# Autodesk Inventor assembly: Soporte filamento
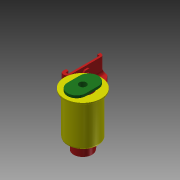
[picture p0: Inventor's stored thumbnail of the model, 180x180]
Saved by Autodesk Inventor 2014 (Build 180170000, 170)
## iProperties
Created: 2017-02-06
Part Number: Soporte filamento
Document SubType Name: Assembly
Designer: Rubén
Author: Rubén
## Documents named in this file (5)
- C:\Users\Rubén\Dropbox\Proyectos\Puma-printer\Piezas Prusa i3 Steel\Soportes filamento\V2\Soporte filamento.iam
- C:\Users\Rubén\Dropbox\Proyectos\Puma-printer\Piezas Prusa i3 Steel\Soportes filamento\V2\Soporte filamento.ipt
- C:\Users\Rubén\Dropbox\Proyectos\Puma-printer\Piezas Prusa i3 Steel\Soportes filamento\V2\Adaptador rollo 5cm.ipt
- C:\Users\Rubén\Dropbox\Proyectos\Puma-printer\Piezas Prusa i3 Steel\Soportes filamento\V2\Cierre.ipt
- C:\Users\Rubén\Dropbox\Proyectos\Puma-printer\Piezas Prusa i3 Steel\Soportes filamento\V2\Cierre V2.ipt
## Components (4 placed, 4 different names)
1. Soporte filamento:1 — Mate:1, Flush:1, Mate:2, Angle:1, Mate:3, Mate:4, Mate:5, Angle:2
2. Adaptador rollo 5cm:1 — Mate:1, Flush:1
3. Cierre:1 — Mate:2, Angle:1, Mate:3
4. Cierre V2:1 — Mate:4, Mate:5, Angle:2
## Relationships (8: Mate 5, Angle 2, Flush 1)
- Mate:1: Soporte filamento:1 ↔ Adaptador rollo 5cm:1
- Flush:1 (1 mm): Soporte filamento:1 ↔ Adaptador rollo 5cm:1
- Mate:2: Soporte filamento:1 ↔ Cierre:1
- Angle:1 (0 deg): Soporte filamento:1 ↔ Cierre:1
- Mate:3: Soporte filamento:1 ↔ Cierre:1
- Mate:4: Soporte filamento:1 ↔ Cierre V2:1
- Mate:5: Soporte filamento:1 ↔ Cierre V2:1
- Angle:2 (0 deg): Soporte filamento:1 ↔ Cierre V2:1
